# Autodesk Inventor assembly: TestBench
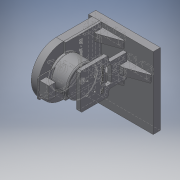
[picture p0: Inventor's stored thumbnail of the model, 180x180]
Saved by Autodesk Inventor 2017 (Build 210142000, 142)
## iProperties
Part Number: TestBench
Material: Générique
Document SubType Name: Assembly
Designer: Darren
Author: Darren
## Documents named in this file (8)
- C:\Users\Darren\Documents\Enseirb\2A_Projet_thematique\Banc de test\TestBench.iam
- C:\Users\Darren\Documents\Enseirb\2A_Projet_thematique\Banc de test\Brushless_70W.ipt
- C:\Users\Darren\Documents\Enseirb\2A_Projet_thematique\Banc de test\Support_motor_front.ipt
- C:\Users\Darren\Documents\Enseirb\2A_Projet_thematique\Banc de test\Support_motor_front_2.ipt
- C:\Users\Darren\Documents\Enseirb\2A_Projet_thematique\Banc de test\Support_motor_front_ground.ipt
- C:\Users\Darren\Documents\Enseirb\2A_Projet_thematique\Banc de test\Support_Carte.ipt
- C:\Users\Darren\Documents\Enseirb\2A_Projet_thematique\Banc de test\Support_carte_ground.ipt
- C:\Users\Darren\Documents\Enseirb\2A_Projet_thematique\Banc de test\Socle_Testbench.ipt
## Components (8 placed, 7 different names)
1. Brushless_70W:1 — Placage:1, Placage:2, Placage:3, Placage:4, Placage:12, Placage:13
2. Support_motor_front:1 — Placage:1, Placage:2, Placage:3, Placage:5, Affleurement:1, Placage:6, Placage:7, Placage:8, Placage:9, Placage:10, Placage:11, Affleurement:2
3. Support_motor_front_2:1 — Placage:4, Placage:5, Affleurement:1
4. Support_motor_front_ground:1 — Placage:6, Placage:7, Placage:8
5. Support_motor_front_ground:2 — Placage:9, Placage:10, Placage:11
6. Support_Carte:1 — Placage:12, Affleurement:2, Placage:13, Placage:14, Placage:15, Placage:16
7. Support_carte_ground:1 — Placage:14, Placage:15, Placage:16, Placage:17, Placage:18, Placage:19
8. Socle_Testbench:1 — Placage:17, Placage:18, Placage:19
## Relationships (21: Mate 19, Flush 2)
- Placage:1 [Mate]: Brushless_70W:1 ↔ Support_motor_front:1
- Placage:2 [Mate]: Brushless_70W:1 ↔ Support_motor_front:1
- Placage:3 [Mate]: Brushless_70W:1 ↔ Support_motor_front:1
- Placage:4 [Mate]: Brushless_70W:1 ↔ Support_motor_front_2:1
- Placage:5 [Mate]: Support_motor_front:1 ↔ Support_motor_front_2:1
- Affleurement:1 [Flush]: Support_motor_front:1 ↔ Support_motor_front_2:1
- Placage:6 [Mate]: Support_motor_front:1 ↔ Support_motor_front_ground:1
- Placage:7 [Mate]: Support_motor_front:1 ↔ Support_motor_front_ground:1
- Placage:8 [Mate]: Support_motor_front:1 ↔ Support_motor_front_ground:1
- Placage:9 [Mate]: Support_motor_front:1 ↔ Support_motor_front_ground:2
- Placage:10 [Mate]: Support_motor_front:1 ↔ Support_motor_front_ground:2
- Placage:11 [Mate]: Support_motor_front:1 ↔ Support_motor_front_ground:2
- Placage:12 [Mate] (6.6 mm): Brushless_70W:1 ↔ Support_Carte:1
- Affleurement:2 [Flush]: Support_motor_front:1 ↔ Support_Carte:1
- Placage:13 [Mate]: Brushless_70W:1 ↔ Support_Carte:1
- Placage:14 [Mate]: Support_Carte:1 ↔ Support_carte_ground:1
- Placage:15 [Mate]: Support_Carte:1 ↔ Support_carte_ground:1
- Placage:16 [Mate]: Support_Carte:1 ↔ Support_carte_ground:1
- Placage:17 [Mate]: Support_carte_ground:1 ↔ Socle_Testbench:1
- Placage:18 [Mate]: Support_carte_ground:1 ↔ Socle_Testbench:1
- Placage:19 [Mate]: Support_carte_ground:1 ↔ Socle_Testbench:1
